# Autodesk Inventor assembly: Baugruppe
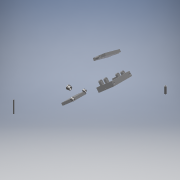
[picture p0: Inventor's stored thumbnail of the model, 180x180]
Saved by Autodesk Inventor 2018.3 (Build 223284000, 284)
## iProperties
Created: 2019-11-29
Part Number: Baugruppe
Material: Generisch
Document SubType Name: Assembly
Designer: maascl
Author: maascl
## Documents named in this file (14)
- U:\MaasCl\IV_13_1\Bauteile_Bohrvorrichtung\Baugruppe.iam
- U:\MaasCl\IV_13_1\Bauteile_Bohrvorrichtung\Anschlag.ipt
- U:\MaasCl\IV_13_1\Bauteile_Bohrvorrichtung\Arretierstift.ipt
- U:\MaasCl\IV_13_1\Bauteile_Bohrvorrichtung\Auswurf.ipt
- U:\MaasCl\IV_13_1\Bauteile_Bohrvorrichtung\Deckel.ipt
- U:\MaasCl\IV_13_1\Bauteile_Bohrvorrichtung\DIN 172 - A 5,5 x 10.ipt
- U:\MaasCl\IV_13_1\Bauteile_Bohrvorrichtung\DIN 172 - A 9,7 x 12.ipt
- U:\MaasCl\IV_13_1\Bauteile_Bohrvorrichtung\DIN 179 - A 5,5 x 10.ipt
- U:\MaasCl\IV_13_1\Bauteile_Bohrvorrichtung\Führungsbock.ipt
- U:\MaasCl\IV_13_1\Bauteile_Bohrvorrichtung\Grundplatte.ipt
- U:\MaasCl\IV_13_1\Bauteile_Bohrvorrichtung\Lagerbock.ipt
- U:\MaasCl\IV_13_1\Bauteile_Bohrvorrichtung\Rändelgriff.ipt
- U:\MaasCl\IV_13_1\Bauteile_Bohrvorrichtung\Stift.ipt
- U:\MaasCl\IV_13_1\Bauteile_Bohrvorrichtung\Werkstück_A.ipt
## Components (13 placed, 13 different names)
1. Anschlag:1 — Passend:8, Passend:9, Passend:10
2. Arretierstift:1
3. Auswurf:1 — Passend:11, Passend:12, Passend:13
4. Deckel:1 — Passend:14, Passend:15
5. DIN 172 - A 5,5 x 10:1
6. DIN 172 - A 9,7 x 12:1
7. DIN 179 - A 5,5 x 10:1
8. Führungsbock:1 — Passend:1, Passend:2, Passend:3, Passend:9, Passend:11
9. Grundplatte:1 — Passend:1, Passend:2, Passend:3, Passend:4, Passend:5, Passend:6, Passend:7, Passend:10, Passend:13, Passend:19
10. Lagerbock:1 — Passend:4, Passend:5, Passend:6, Passend:7, Passend:8, Passend:12
11. Rändelgriff:1
12. Stift:1 — Passend:14, Passend:15
13. Werkstück_A:1 — Passend:19
## Relationships (16: Mate 16)
- Passend:1 [Mate]: Führungsbock:1 ↔ Grundplatte:1
- Passend:2 [Mate]: Führungsbock:1 ↔ Grundplatte:1
- Passend:3 [Mate]: Führungsbock:1 ↔ Grundplatte:1
- Passend:4 [Mate]: Grundplatte:1 ↔ Lagerbock:1
- Passend:5 [Mate]: Grundplatte:1 ↔ Lagerbock:1
- Passend:6 [Mate]: Grundplatte:1 ↔ Lagerbock:1
- Passend:7 [Mate]: Grundplatte:1 ↔ Lagerbock:1
- Passend:8 [Mate]: Anschlag:1 ↔ Lagerbock:1
- Passend:9 [Mate]: Anschlag:1 ↔ Führungsbock:1
- Passend:10 [Mate]: Anschlag:1 ↔ Grundplatte:1
- Passend:11 [Mate]: Auswurf:1 ↔ Führungsbock:1
- Passend:12 [Mate]: Auswurf:1 ↔ Lagerbock:1
- Passend:13 [Mate]: Auswurf:1 ↔ Grundplatte:1
- Passend:14 [Mate]: Deckel:1 ↔ Stift:1
- Passend:15 [Mate]: Deckel:1 ↔ Stift:1
- Passend:19 [Mate]: Grundplatte:1 ↔ Werkstück_A:1
